# Autodesk Inventor assembly: XEndRight
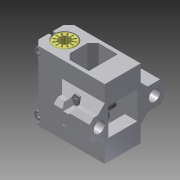
[picture p0: Inventor's stored thumbnail of the model, 180x180]
Saved by Autodesk Inventor 2015 (Build 190159000, 159)
## iProperties
Created: 2014-08-10
Part Number: XEndRight
Document SubType Name: Assembly
Designer: Jack
Author: Jack
## Documents named in this file (9)
- C:\Users\Jack\ownCloud\Projects\CoreXY\InventorModel\XAxis\XEndRight.iam
- C:\Users\Jack\ownCloud\Projects\CoreXY\InventorModel\XAxis\XEnd.ipt
- C:\Users\Jack\ownCloud\Projects\CoreXY\InventorModel\Hardware\Bolts\SHCS\SHCS4\SHCS4x30.ipt
- C:\Users\Jack\ownCloud\Projects\CoreXY\InventorModel\Hardware\Nuts\Nut4.ipt
- C:\Users\Jack\ownCloud\Projects\CoreXY\InventorModel\Hardware\Wahsers\M4Washer.ipt
- C:\Users\Jack\ownCloud\Projects\CoreXY\InventorModel\Hardware\Bearings \Igus\BushingIgusRJM-01-08.ipt
- C:\Users\Jack\ownCloud\Projects\CoreXY\InventorModel\Hardware\Bolts\SHCS\SHCS3\SHCS3x25.ipt
- C:\Users\Jack\ownCloud\Projects\CoreXY\InventorModel\Hardware\Nuts\Nut3.ipt
- C:\Users\Jack\ownCloud\Projects\CoreXY\InventorModel\Hardware\Bearings \BearingRadialBall\BearingRadialBallF624zz.ipt
## Components (20 placed, 8 different names)
1. XEnd:1 — Mate:6, Mate:7, Mate:8, Mate:9, Mate:11, Angle:1, Mate:13, Angle:2, Mate:25, Flush:1, Flush:2, Mate:38, Mate:39, Mate:42, Mate:43, Mate:44, Mate:45, Mate:48, Mate:49, Angle:3, Angle:4, Mate:64, Mate:65
2. SHCS4x30:1 — Mate:7, Mate:9, Mate:12, Mate:36, Mate:63
3. SHCS4x30:2 — Mate:6, Mate:8, Mate:10, Mate:62
4. Nut4:1 — Mate:10, Mate:11, Angle:1
5. Nut4:2 — Mate:12, Mate:13, Angle:2
6. M4Washer:3 — Mate:36
7. BushingIgusRJM-01-08:1 — Mate:38
8. BushingIgusRJM-01-08:2 — Mate:39
9. SHCS3x25:1 — Mate:42, Mate:44, Mate:47
10. SHCS3x25:2 — Mate:43, Mate:45, Mate:46
11. Nut3:1 — Mate:47, Mate:48, Angle:4
12. Nut3:2 — Mate:46, Mate:49, Angle:3
13. BearingRadialBallF624zz:1
14. BearingRadialBallF624zz:2
15. M4Washer:4
16. M4Washer:5 — Mate:62, Mate:65
17. BearingRadialBallF624zz:3
18. BearingRadialBallF624zz:4
19. M4Washer:6
20. M4Washer:7 — Mate:63, Mate:64
## Relationships (42: Mate 36, Angle 4, Flush 2)
- Mate:6: XEnd:1 ↔ SHCS4x30:2
- Mate:7: XEnd:1 ↔ SHCS4x30:1
- Mate:8: XEnd:1 ↔ SHCS4x30:2
- Mate:9: XEnd:1 ↔ SHCS4x30:1
- Mate:10: SHCS4x30:2 ↔ Nut4:1
- Mate:11: XEnd:1 ↔ Nut4:1
- Angle:1 (0 deg): XEnd:1 ↔ Nut4:1
- Mate:12: SHCS4x30:1 ↔ Nut4:2
- Mate:13: XEnd:1 ↔ Nut4:2
- Angle:2 (0 deg): XEnd:1 ↔ Nut4:2
- Mate:25: XEnd:1
- Flush:1: XEnd:1
- Flush:2: XEnd:1
- Mate:36: SHCS4x30:1 ↔ M4Washer:3
- Mate:38: XEnd:1 ↔ BushingIgusRJM-01-08:1
- Mate:39: XEnd:1 ↔ BushingIgusRJM-01-08:2
- Mate:42: XEnd:1 ↔ SHCS3x25:1
- Mate:43: XEnd:1 ↔ SHCS3x25:2
- Mate:44: XEnd:1 ↔ SHCS3x25:1
- Mate:45: XEnd:1 ↔ SHCS3x25:2
- Mate:46: SHCS3x25:2 ↔ Nut3:2
- Mate:47: SHCS3x25:1 ↔ Nut3:1
- Mate:48: XEnd:1 ↔ Nut3:1
- Mate:49: XEnd:1 ↔ Nut3:2
- Angle:3 (0 deg): XEnd:1 ↔ Nut3:2
- Angle:4 (0 deg): XEnd:1 ↔ Nut3:1
- [Mate]: BearingRadialBallF624zz:1 ↔ BearingRadialBallF624zz:2
- [Mate]: BearingRadialBallF624zz:1 ↔ BearingRadialBallF624zz:2
- [Mate]: BearingRadialBallF624zz:1 ↔ M4Washer:4
- [Mate]: BearingRadialBallF624zz:2 ↔ M4Washer:4
- [Mate]: BearingRadialBallF624zz:1 ↔ M4Washer:5
- [Mate]: BearingRadialBallF624zz:1 ↔ M4Washer:5
- [Mate]: BearingRadialBallF624zz:3 ↔ BearingRadialBallF624zz:4
- [Mate]: BearingRadialBallF624zz:3 ↔ BearingRadialBallF624zz:4
- [Mate]: BearingRadialBallF624zz:3 ↔ M4Washer:6
- [Mate]: BearingRadialBallF624zz:4 ↔ M4Washer:6
- [Mate]: BearingRadialBallF624zz:3 ↔ M4Washer:7
- [Mate]: BearingRadialBallF624zz:3 ↔ M4Washer:7
- Mate:62: SHCS4x30:2 ↔ M4Washer:5
- Mate:63: SHCS4x30:1 ↔ M4Washer:7
- Mate:64: XEnd:1 ↔ M4Washer:7
- Mate:65: XEnd:1 ↔ M4Washer:5
## Named parameters: d64_d160 = 0 mm, d65_d161 = 0 mm, d66_d162 = 0 mm, d67_d163 = 0 mm, d68_d158 = 0 mm, d69_d159 = 0 mm
